# Autodesk Inventor assembly: Hinge_p1_assembly
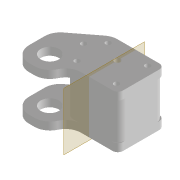
[picture p0: Inventor's stored thumbnail of the model, 180x180]
Saved by Autodesk Inventor 2022 (Build 260153000, 153)
## iProperties
Created: 2022-07-11
Part Number: Hinge_p1_assembly
Document SubType Name: Assembly
Designer: dell
Author: dell
## Documents named in this file (3)
- D:\xxxx\Uni\Part IV\MECHENG_700\Part_IV_project_CAD\Bird_skeleton_prototypes\Wing_drone_V1\Bird_wing_V2\Hinge_p1_assembly.iam
- D:\xxxx\Uni\Part IV\MECHENG_700\Part_IV_project_CAD\Bird_skeleton_prototypes\Wing_drone_V1\Bird_wing_V2\Hinge_p1.ipt
- D:\xxxx\Uni\Part IV\MECHENG_700\Part_IV_project_CAD\Bird_skeleton_prototypes\Wing_drone_V1\Bird_wing_V2\Hinge_p1_plate.ipt
## Components (3 placed, 2 different names)
1. Hinge_p1:1 — Mate:1, Mate:2, Mate:3, Mate:4, Mate:5, Mate:6
2. Hinge_p1_plate:1 — Mate:1, Mate:5, Mate:6
3. Hinge_p1_plate:2 — Mate:2, Mate:3, Mate:4
## Relationships (6: Mate 6)
- Mate:1: Hinge_p1:1 ↔ Hinge_p1_plate:1
- Mate:2: Hinge_p1:1 ↔ Hinge_p1_plate:2
- Mate:3: Hinge_p1:1 ↔ Hinge_p1_plate:2
- Mate:4: Hinge_p1:1 ↔ Hinge_p1_plate:2
- Mate:5: Hinge_p1:1 ↔ Hinge_p1_plate:1
- Mate:6: Hinge_p1:1 ↔ Hinge_p1_plate:1
